# Autodesk Inventor assembly: EncoderV2.5_MIR
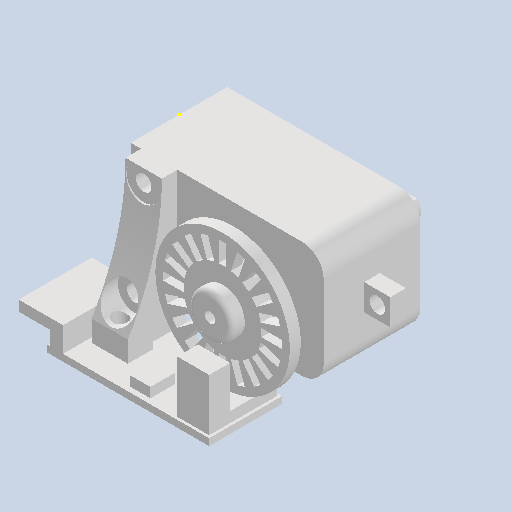
[picture p0: Inventor's stored thumbnail of the model, 512x512]
Saved by Autodesk Inventor 2022 (Build 260153070, 153G)
## iProperties
Created: 2022-01-31
Part Number: EncoderV2.5_MIR
Document SubType Name: Assembly
Designer: a laptop
Author: a laptop
## Documents named in this file (7)
- C:\Users\a laptop\Desktop\SumoBot\sumobotENCODER\EncoderV2\EncoderV2.5_MIR.iam
- C:\Users\a laptop\Desktop\SumoBot\sumobotENCODER\REF_PART\LM393 encoder_MIR1.ipt
- C:\Users\a laptop\Desktop\SumoBot\sumobotENCODER\REF_PART\TT encoder disk_MIR1.ipt
- C:\Users\a laptop\Desktop\SumoBot\sumobotENCODER\REF_PART\TT motor output_MIR1.ipt
- C:\Users\a laptop\Desktop\SumoBot\sumobotENCODER\REF_PART\TTencoderspacer_MIR1.ipt
- C:\Users\a laptop\Desktop\SumoBot\sumobotENCODER\EncoderV2\EncoderV2CAP_MIR.ipt
- C:\Users\a laptop\Desktop\SumoBot\sumobotENCODER\EncoderV2\ENCODERV2PLATE_MIR.ipt
## Components (6 placed, 6 different names)
1. LM393 encoder_MIR1:1 — Mate:12, Mate:8
2. TT encoder disk_MIR1:1 — Mate:5, Mate:4, Mate:3, Mate:6
3. TT motor output_MIR1:1 — Mate:5, Mate:4, Mate:2, Mate:1, Mate:7, Mate:11, Mate:10, Mate:9
4. TTencoderspacer_MIR1:1 — Mate:3, Mate:2, Mate:1
5. EncoderV2CAP_MIR:1 — Mate:7, Mate:6
6. ENCODERV2PLATE_MIR:1 — Mate:12, Mate:11, Mate:10, Mate:9, Mate:8
## Relationships (12: Mate 12)
- Mate:5: TT encoder disk_MIR1:1 ↔ TT motor output_MIR1:1
- Mate:4: TT encoder disk_MIR1:1 ↔ TT motor output_MIR1:1
- Mate:3: TT encoder disk_MIR1:1 ↔ TTencoderspacer_MIR1:1
- Mate:2: TT motor output_MIR1:1 ↔ TTencoderspacer_MIR1:1
- Mate:1: TT motor output_MIR1:1 ↔ TTencoderspacer_MIR1:1
- Mate:7: TT motor output_MIR1:1 ↔ EncoderV2CAP_MIR:1
- Mate:6: TT encoder disk_MIR1:1 ↔ EncoderV2CAP_MIR:1
- Mate:12: LM393 encoder_MIR1:1 ↔ ENCODERV2PLATE_MIR:1
- Mate:11: TT motor output_MIR1:1 ↔ ENCODERV2PLATE_MIR:1
- Mate:10: TT motor output_MIR1:1 ↔ ENCODERV2PLATE_MIR:1
- Mate:9: TT motor output_MIR1:1 ↔ ENCODERV2PLATE_MIR:1
- Mate:8: LM393 encoder_MIR1:1 ↔ ENCODERV2PLATE_MIR:1
